# Autodesk Inventor assembly: MechanismAssembly
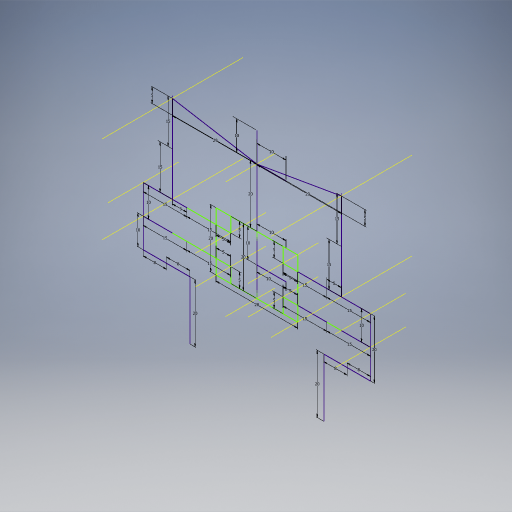
[picture p0: Inventor's stored thumbnail of the model, 512x512]
Saved by Autodesk Inventor 2024.1 (Build 281209000, 209)
## iProperties
Created: 2023-09-08
Part Number: MechanismAssembly
Document SubType Name: Assembly
Designer: Camilo
Author: Camilo
## Documents named in this file (12)
- D:\Documentos\MEGA\Universidad\2023-2\Dinamica Computacional de Sistemas Multicuerpo\DinamicaComputacionalSistemasMulticuerpo\Proyecto\CAD\2D\MechanismAssembly.iam
- D:\Documentos\MEGA\Universidad\2023-2\Dinamica Computacional de Sistemas Multicuerpo\DinamicaComputacionalSistemasMulticuerpo\Proyecto\CAD\2D\link1.ipt
- D:\Documentos\MEGA\Universidad\2023-2\Dinamica Computacional de Sistemas Multicuerpo\DinamicaComputacionalSistemasMulticuerpo\Proyecto\CAD\2D\link2.ipt
- D:\Documentos\MEGA\Universidad\2023-2\Dinamica Computacional de Sistemas Multicuerpo\DinamicaComputacionalSistemasMulticuerpo\Proyecto\CAD\2D\link3.ipt
- D:\Documentos\MEGA\Universidad\2023-2\Dinamica Computacional de Sistemas Multicuerpo\DinamicaComputacionalSistemasMulticuerpo\Proyecto\CAD\2D\link4.ipt
- D:\Documentos\MEGA\Universidad\2023-2\Dinamica Computacional de Sistemas Multicuerpo\DinamicaComputacionalSistemasMulticuerpo\Proyecto\CAD\2D\link5.ipt
- D:\Documentos\MEGA\Universidad\2023-2\Dinamica Computacional de Sistemas Multicuerpo\DinamicaComputacionalSistemasMulticuerpo\Proyecto\CAD\2D\link6.ipt
- D:\Documentos\MEGA\Universidad\2023-2\Dinamica Computacional de Sistemas Multicuerpo\DinamicaComputacionalSistemasMulticuerpo\Proyecto\CAD\2D\link8.ipt
- D:\Documentos\MEGA\Universidad\2023-2\Dinamica Computacional de Sistemas Multicuerpo\DinamicaComputacionalSistemasMulticuerpo\Proyecto\CAD\2D\link9.ipt
- D:\Documentos\MEGA\Universidad\2023-2\Dinamica Computacional de Sistemas Multicuerpo\DinamicaComputacionalSistemasMulticuerpo\Proyecto\CAD\2D\link7.ipt
- D:\Documentos\MEGA\Universidad\2023-2\Dinamica Computacional de Sistemas Multicuerpo\DinamicaComputacionalSistemasMulticuerpo\Proyecto\CAD\2D\link11.ipt
- D:\Documentos\MEGA\Universidad\2023-2\Dinamica Computacional de Sistemas Multicuerpo\DinamicaComputacionalSistemasMulticuerpo\Proyecto\CAD\2D\link10.ipt
## Components (11 placed, 11 different names)
1. link1:1 — Rotation:1
2. link2:1 — Rotation:1
3. link3:1
4. link4:1
5. link5:1
6. link6:1
7. link8:1
8. link9:1
9. link7:1
10. link11:1
11. link10:1
## Relationships (1: RelateRotation 1)
- Rotation:1 [RelateRotation] (1 ul): link1:1 ↔ link2:1
